# Autodesk Inventor assembly: Outer Channel
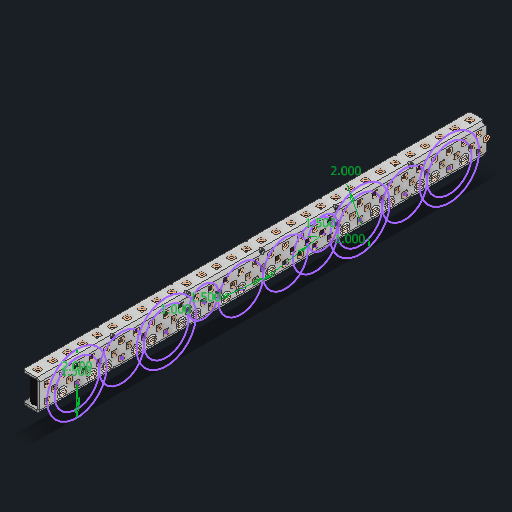
[picture p0: Inventor's stored thumbnail of the model, 512x512]
Saved by Autodesk Inventor 2025.1 (Build 291241000, 241)
## iProperties
Created: 2024-11-04
Part Number: Outer Channel
Document SubType Name: Assembly
Designer: avere
Author: avere
## Documents named in this file (5)
- C:\Users\avere\VEX\High Stakes\CAD\V3\Chassis\Drivebay Left\Outer Channel.iam
- C:\Users\avere\VEX\High Stakes\CAD\ROBOPROS-CAD-Inventor\Structure\C Channel\Aluminum 1x2x1\Alu C 1x2x1x30.ipt
- C:\Users\avere\VEX\High Stakes\CAD\ROBOPROS-CAD-Inventor\Quick Assemblies\Bearing Flat NScrew Slotted.iam
- C:\Users\avere\VEX\High Stakes\CAD\ROBOPROS-CAD-Inventor\Motion\Spacers\Spacer Nylon .375 OD\NSpacer .375 OD x .875.ipt
- C:\Users\avere\VEX\High Stakes\CAD\ROBOPROS-CAD-Inventor\Motion\Spacers\Spacer Nylon .375 OD.ipt
## Components (10 placed, 3 different names)
1. Alu C 1x2x1x30:1 — Flush:1, Flush:2, Flush:3, Insert:7, Mate:7, Insert:8, Mate:8, Insert:9
2. NSpacer .375 OD x .875:1 — Insert:9
3. Bearing Flat NScrew Slotted:8 [sub-assembly] — Insert:7, Mate:7
4. Bearing Flat NScrew Slotted:9 [sub-assembly]
5. Bearing Flat NScrew Slotted:10 [sub-assembly]
6. Bearing Flat NScrew Slotted:11 [sub-assembly]
7. Bearing Flat NScrew Slotted:12 [sub-assembly]
8. Bearing Flat NScrew Slotted:13 [sub-assembly] — Insert:8, Mate:8
9. Bearing Flat NScrew Slotted:14 [sub-assembly]
10. Bearing Flat NScrew Slotted:15 [sub-assembly]
## Component patterns: Front Bearings (5 elements), Back Bearings (3 elements)
## Relationships (8: Flush 3, Insert 3, Mate 2)
- Flush:1 (-190.5 mm): Alu C 1x2x1x30:1
- Flush:2 (-12.7 mm): Alu C 1x2x1x30:1
- Flush:3 (-7.9375 mm): Alu C 1x2x1x30:1
- Insert:7: Alu C 1x2x1x30:1 ↔ Bearing Flat NScrew Slotted:8
- Mate:7: Alu C 1x2x1x30:1 ↔ Bearing Flat NScrew Slotted:8
- Insert:8: Alu C 1x2x1x30:1 ↔ Bearing Flat NScrew Slotted:13
- Mate:8: Alu C 1x2x1x30:1 ↔ Bearing Flat NScrew Slotted:13
- Insert:9: Alu C 1x2x1x30:1 ↔ NSpacer .375 OD x .875:1
